# Autodesk Inventor assembly: Calorimeter with test
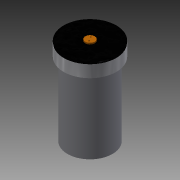
[picture p0: Inventor's stored thumbnail of the model, 180x180]
Saved by Autodesk Inventor 2014 (Build 180170000, 170)
## iProperties
Created: 2014-06-11
Part Number: Calorimeter with test
Document SubType Name: Assembly
Designer: Nabeel
Author: Nabeel
## Documents named in this file (6)
- C:\Users\Nabeel\Desktop\Nabu Stuff\VERL Work\Calorimeter\Calorimeter with test.iam
- C:\Users\Nabeel\Desktop\Nabu Stuff\VERL Work\Calorimeter\Outter Cup.ipt
- C:\Users\Nabeel\Desktop\Nabu Stuff\VERL Work\Calorimeter\Inner Cup.ipt
- C:\Users\Nabeel\Desktop\Nabu Stuff\VERL Work\Calorimeter\Plastic Lid.ipt
- C:\Users\Nabeel\Desktop\Nabu Stuff\VERL Work\Calorimeter\Rubber Stopper.ipt
- C:\Users\Nabeel\Desktop\Nabu Stuff\VERL Work\Specific heat set\Brass.ipt
## Components (5 placed, 5 different names)
1. Outter Cup:1 — Mate:1, Mate:3, Mate:5
2. Inner Cup:1 — Mate:1, Mate:4
3. Plastic Lid:1 — Mate:3, Mate:5, Mate:6
4. Rubber Stopper:1 — Mate:6
5. Brass:1 — Mate:4
## Relationships (5: Mate 5)
- Mate:1: Outter Cup:1 ↔ Inner Cup:1
- Mate:3: Outter Cup:1 ↔ Plastic Lid:1
- Mate:4: Inner Cup:1 ↔ Brass:1
- Mate:5: Outter Cup:1 ↔ Plastic Lid:1
- Mate:6: Plastic Lid:1 ↔ Rubber Stopper:1
